# Autodesk Inventor assembly: 足ユニット
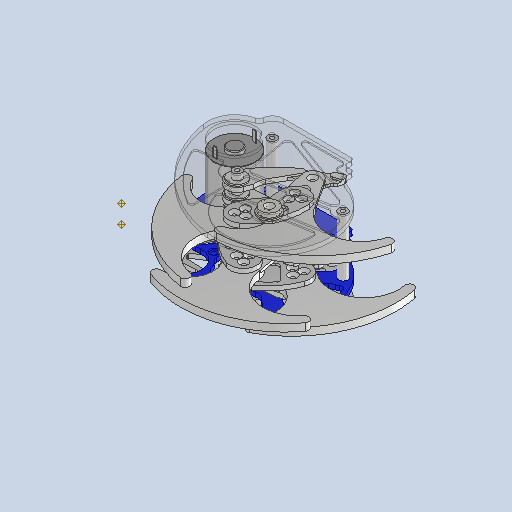
[picture p0: Inventor's stored thumbnail of the model, 512x512]
Saved by Autodesk Inventor 2023 (Build 270158030, 158C)
## iProperties
Created: 2022-01-10
Part Number: 足ユニット
Document SubType Name: Assembly
Designer: acps
Mass: 295.888 g
Surface Area: 1084.8 cm^2
Volume: 133.422 cm^3
Density: 2.21768 g/cm^3
Author: acps
## Documents named in this file (21)
- C:\Users\muzho\Documents\srdc\srdc_2\脚\足ユニット.iam
- C:\Users\muzho\Documents\srdc\srdc_2\脚\足外フレーム.ipt
- C:\Users\muzho\Documents\srdc\srdc_2\脚\足内フレーム.ipt
- C:\Users\muzho\Documents\srdc\srdc_2\スペーサ\l40.ipt
- C:\Users\muzho\Documents\srdc\srdc_2\カム\カム4.ipt
- C:\Users\muzho\Documents\srdc\srdc_2\オイレス\w5f15-17n.ipt
- C:\Users\muzho\Documents\srdc\srdc_2\モータ\M-RS-380.ipt
- C:\Users\muzho\Documents\srdc\srdc_2\脚\モータマウント.ipt
- C:\Users\muzho\Documents\srdc\srdc_2\ベアリング\φ6φ12ベアリングa.ipt
- C:\Users\muzho\Documents\srdc\srdc_2\脚\ギア\初段_多段ギア.iam
- C:\Users\muzho\Documents\srdc\srdc_2\脚\ギア\ぴにょん.ipt
- C:\Users\muzho\Documents\srdc\srdc_2\ベアリング\M-φ4φ8a.ipt
- C:\Users\muzho\Documents\srdc\srdc_2\ベアリング\φ4φ8ベアリングa.ipt
- C:\Users\muzho\Documents\srdc\srdc_2\脚\ギア\最終段m2z28t4.ipt
- C:\Users\muzho\Documents\srdc\srdc_2\脚\クランク.iam
- C:\Users\muzho\Documents\srdc\srdc_2\脚\揺動節+ヘッケン.iam
- C:\Users\muzho\Documents\srdc\srdc_2\スペーサ\l14.ipt
- C:\Users\muzho\Documents\srdc\srdc_2\脚\ギア抑え.ipt
- C:\Users\muzho\Documents\srdc\srdc_2\ベアリング\φ6φ10ベアリングa.ipt
- C:\Users\muzho\Documents\srdc\srdc_2\ピン\φ4l20.ipt
- C:\Users\muzho\Documents\srdc\srdc_2\オイレス\w6f15-17a.ipt
## Components (31 placed, 20 different names)
1. l40:1 — Insert:68, 挿入:89
2. l40:2 — Insert:67
3. l40:3 — Mate:49, Mate:51, Mate:53, Mate:55, Mate:64, Insert:65
4. カム4:1 — Insert:9, Insert:51, Mate:68, Mate:69, Mate:70, Insert:75
5. w5f15-17n:1 — Insert:9
6. M-RS-380:1 — Insert:31, Mate:38, Insert:32, Mate:61, Mate:62, Mate:71
7. φ6φ12ベアリングa:1 — Insert:86, 挿入:90
8. モータマウント:1 — Insert:31, Mate:61, Mate:71, Insert:83, Mate:76
9. ぴにょん:1 — Mate:38, Insert:32
10. M-φ4φ8a:1 — Mate:41, Mate:77, Insert:87, 挿入:97
11. 初段_多段ギア:1 [sub-assembly] — Mate:41, Mate:62
12. φ4φ8ベアリングa:1
13. 最終段m2z28t4:1 — Mate:69, Mate:70, Insert:75, メイト:78, メイト:79, 挿入:88
14. クランク:1 [sub-assembly] — Insert:51, Mate:50, Insert:52, Mate:52, Insert:54, Mate:54, Insert:55, Mate:56, Insert:56, Mate:68, 挿入:90
15. 揺動節+ヘッケン:1 [sub-assembly] — Mate:51, Mate:52, Insert:54
16. 揺動節+ヘッケン:2 [sub-assembly] — Mate:53, Mate:54, Insert:55
17. 揺動節+ヘッケン:3 [sub-assembly] — Mate:55, Mate:56, Insert:56
18. 揺動節+ヘッケン:4 [sub-assembly] — Mate:49, Mate:50, Insert:52
19. l14:1
20. l14:2 — Insert:82
21. l14:3 — 挿入:93, 挿入:96
22. 足外フレーム:1 — Mate:64, Insert:65, Insert:67, Insert:68, Mate:74, Mate:75, Insert:86
23. ギア抑え:1 — メイト:84, 挿入:96, 挿入:97
24. 足内フレーム:1 — Mate:74, Mate:75, Insert:82, Insert:83, Mate:76, Insert:85, 挿入:89, 挿入:93, 挿入:95
25. φ6φ10ベアリングa:1
26. φ6φ10ベアリングa:2 — Insert:85
27. φ4l20:1 — Mate:77, Insert:87
28. カム4:2 — メイト:78, メイト:79, 挿入:88, メイト:82, メイト:83, 挿入:92
29. w6f15-17a:1
30. カム4:3 — メイト:82, メイト:83, 挿入:92
31. l14:4 — 挿入:95, メイト:84
## Relationships (51: Mate 26, Insert 25)
- Insert:9: カム4:1 ↔ w5f15-17n:1
- Insert:31: M-RS-380:1 ↔ モータマウント:1
- Mate:38: M-RS-380:1 ↔ ぴにょん:1
- Insert:32: M-RS-380:1 ↔ ぴにょん:1
- Mate:41: M-φ4φ8a:1 ↔ 初段_多段ギア:1
- Insert:51: カム4:1 ↔ クランク:1
- Mate:49: l40:3 ↔ 揺動節+ヘッケン:4
- Mate:50: クランク:1 ↔ 揺動節+ヘッケン:4
- Insert:52 (0.25 mm): クランク:1 ↔ 揺動節+ヘッケン:4
- Mate:51: l40:3 ↔ 揺動節+ヘッケン:1
- Mate:52: クランク:1 ↔ 揺動節+ヘッケン:1
- Insert:54 (0.25 mm): クランク:1 ↔ 揺動節+ヘッケン:1
- Mate:53: l40:3 ↔ 揺動節+ヘッケン:2
- Mate:54: クランク:1 ↔ 揺動節+ヘッケン:2
- Insert:55 (0.25 mm): クランク:1 ↔ 揺動節+ヘッケン:2
- Mate:55: l40:3 ↔ 揺動節+ヘッケン:3
- Mate:56: クランク:1 ↔ 揺動節+ヘッケン:3
- Insert:56 (0.25 mm): クランク:1 ↔ 揺動節+ヘッケン:3
- Mate:61: M-RS-380:1 ↔ モータマウント:1
- Mate:62 (0.3 mm): M-RS-380:1 ↔ 初段_多段ギア:1
- Mate:64: l40:3 ↔ 足外フレーム:1
- Insert:65: l40:3 ↔ 足外フレーム:1
- Insert:67: l40:2 ↔ 足外フレーム:1
- Insert:68: l40:1 ↔ 足外フレーム:1
- Mate:68: カム4:1 ↔ クランク:1
- Mate:69: カム4:1 ↔ 最終段m2z28t4:1
- Mate:70: カム4:1 ↔ 最終段m2z28t4:1
- Insert:75: カム4:1 ↔ 最終段m2z28t4:1
- Mate:71: M-RS-380:1 ↔ モータマウント:1
- Mate:74: 足外フレーム:1 ↔ 足内フレーム:1
- Mate:75: 足外フレーム:1 ↔ 足内フレーム:1
- Insert:82: l14:2 ↔ 足内フレーム:1
- Insert:83: モータマウント:1 ↔ 足内フレーム:1
- Mate:76: モータマウント:1 ↔ 足内フレーム:1
- Insert:85: 足内フレーム:1 ↔ φ6φ10ベアリングa:2
- Insert:86: φ6φ12ベアリングa:1 ↔ 足外フレーム:1
- Mate:77: M-φ4φ8a:1 ↔ φ4l20:1
- Insert:87 (0.5 mm): M-φ4φ8a:1 ↔ φ4l20:1
- メイト:78 [Mate]: 最終段m2z28t4:1 ↔ カム4:2
- メイト:79 [Mate]: 最終段m2z28t4:1 ↔ カム4:2
- 挿入:88 [Insert]: 最終段m2z28t4:1 ↔ カム4:2
- 挿入:89 [Insert]: l40:1 ↔ 足内フレーム:1
- 挿入:90 [Insert]: φ6φ12ベアリングa:1 ↔ クランク:1
- メイト:82 [Mate]: カム4:2 ↔ カム4:3
- メイト:83 [Mate]: カム4:2 ↔ カム4:3
- 挿入:92 [Insert]: カム4:2 ↔ カム4:3
- 挿入:93 [Insert]: l14:3 ↔ 足内フレーム:1
- 挿入:95 [Insert]: 足内フレーム:1 ↔ l14:4
- メイト:84 [Mate]: ギア抑え:1 ↔ l14:4
- 挿入:96 [Insert]: l14:3 ↔ ギア抑え:1
- 挿入:97 [Insert]: M-φ4φ8a:1 ↔ ギア抑え:1
